# Autodesk Inventor assembly: 4xSplitter
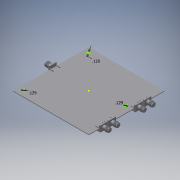
[picture p0: Inventor's stored thumbnail of the model, 180x180]
Saved by Autodesk Inventor 2018 (Build 220112000, 112)
## iProperties
Created: 2018-04-06
Part Number: 4xSplitter
Document SubType Name: Assembly
Designer: bbramman
Author: bbramman
## Documents named in this file (3)
- C:\Users\bbramman\OneDrive\Documents\Trapped Ion Research (Grad)\Electronics\pll-evalboard-synthesizer\Box CAD\4xSplitter.iam
- C:\Users\bbramman\OneDrive\Documents\Trapped Ion Research (Grad)\Electronics\pll-evalboard-synthesizer\Box CAD\4xSplitter.ipt
- C:\Users\bbramman\OneDrive\Documents\Trapped Ion Research (Grad)\Electronics\pll-evalboard-synthesizer\Box CAD\SMA-END.ipt
## Components (6 placed, 2 different names)
1. 4xSplitter:1 — Mate:1, Mate:2, Flush:1, Mate:3, Mate:4, Mate:5, Mate:6, Mate:7, Mate:8, Mate:9, Mate:10
2. SMA-END:1 — Mate:1, Mate:2, Flush:1
3. SMA-END:2 — Mate:3, Mate:4
4. SMA-END:3 — Mate:5, Mate:6
5. SMA-END:4 — Mate:9, Mate:10
6. SMA-END:5 — Mate:7, Mate:8
## Relationships (11: Mate 10, Flush 1)
- Mate:1: 4xSplitter:1 ↔ SMA-END:1
- Mate:2: 4xSplitter:1 ↔ SMA-END:1
- Flush:1 (48.26 mm): 4xSplitter:1 ↔ SMA-END:1
- Mate:3: 4xSplitter:1 ↔ SMA-END:2
- Mate:4: 4xSplitter:1 ↔ SMA-END:2
- Mate:5: 4xSplitter:1 ↔ SMA-END:3
- Mate:6: 4xSplitter:1 ↔ SMA-END:3
- Mate:7: 4xSplitter:1 ↔ SMA-END:5
- Mate:8: 4xSplitter:1 ↔ SMA-END:5
- Mate:9: 4xSplitter:1 ↔ SMA-END:4
- Mate:10: 4xSplitter:1 ↔ SMA-END:4
